# Autodesk Inventor assembly: Driveopen2
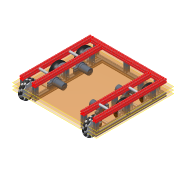
[picture p0: Inventor's stored thumbnail of the model, 180x180]
Saved by Autodesk Inventor 2013 (Build 170138000, 138)
## iProperties
Created: 2013-09-22
Part Number: Driveopen2
Document SubType Name: Assembly
Designer: Family Room
Mass: 858.54 g
Surface Area: 8628.43 cm^2
Volume: 788.69 cm^3
Density: 1.08856 g/cm^3
Author: Family Room
## Documents named in this file (14)
- H:\Driveopen2.iam
- H:\Frame Layer open.iam
- H:\Verticle support.ipt
- C:\Users\Family Room\Documents\Inventor\Content Center Files\R2011\en-US\ANSI B18.3(13)\ANSI B18.3 - 1_4-28 UNF - 1(22).ipt
- H:\axel support.ipt
- H:\Tetrix Wheel 4 in omni.ipt
- H:\Tetrix wheel 4 in.ipt
- H:\pvc holder.ipt
- C:\Users\rihoobler\Documents\Inventor\tetrix_739091_2012.ipt
- U:\Imported Components\tetrix_739088_2012\tetrix_739088_2012.ipt
- U:\Imported Components\tetrix_739165_2012\tetrix_739165_2012.ipt
- U:\Imported Components\tetrix_739172_2012\tetrix_739172_2012.iam
- H:\Motor Mount.ipt
- H:\Motor.iam
## Components (81 placed, 13 different names)
1. Frame Layer open:1 [sub-assembly] — Mate:3, Flush:5, Mate:4, Flush:6, Flush:9, Mate:6, Flush:11, Insert:4, Insert:5, Insert:6, Mate:12, Flush:12, Flush:13, Mate:13, Flush:14, Flush:15, Mate:14, Flush:16, Flush:17, Mate:15, Angle:1, Flush:18, Mate:17, Angle:2, Mate:18, Mate:19, Flush:19, Mate:20, Flush:21, Mate:21, Flush:23, Flush:24, Mate:22, Flush:25, Mate:23, Flush:27, Mate:24, Flush:29, Mate:25, Flush:31, Mate:32, Mate:35, Mate:37, Mate:38, Flush:44, Mate:72, Flush:50, Mate:74, Flush:51, Mate:76, Flush:52, Flush:53, Mate:77, Flush:60
2. Frame Layer open:2 [sub-assembly] — Flush:9, Flush:10, Insert:1, Insert:2, Insert:3, Mate:33, Mate:34, Mate:36, Mate:39
3. Verticle support:3 — Mate:4, Flush:6, Flush:10, Mate:7, Mate:10
4. Verticle support:4 — Mate:3, Flush:5, Mate:11
5. Verticle support:5 — Mate:6, Flush:11, Mate:7
6. Spline Socket Head Cap Screw - Inch 1/4-28 UNF - 1:1 — Insert:1
7. Spline Socket Head Cap Screw - Inch 1/4-28 UNF - 1:2 — Insert:2
8. Spline Socket Head Cap Screw - Inch 1/4-28 UNF - 1:3 — Insert:3
9. Spline Socket Head Cap Screw - Inch 1/4-28 UNF - 1:4 — Insert:4, Mate:10
10. Spline Socket Head Cap Screw - Inch 1/4-28 UNF - 1:5 — Insert:5
11. Spline Socket Head Cap Screw - Inch 1/4-28 UNF - 1:6 — Insert:6, Mate:11
12. axel support:1 — Mate:14, Flush:16, Flush:17, Mate:27, Insert:7
13. axel support:2 — Mate:25, Flush:31, Flush:32, Mate:31, Mate:48, Flush:43
14. axel support:3 — Mate:21, Flush:23, Flush:24, Mate:46, Mate:49, Flush:41
15. axel support:4 — Mate:12, Flush:12, Flush:13, Mate:16, Mate:26, Insert:10
16. axel support:5 — Mate:13, Flush:14, Flush:15, Insert:11, Flush:40
17. axel support:6 — Mate:15, Angle:1, Flush:18, Mate:16, Flush:20, Flush:26, Mate:28, Insert:14, Mate:73
18. axel support:7 — Mate:17, Angle:2, Mate:18, Flush:22, Flush:28, Mate:29, Insert:15, Mate:75
19. axel support:8 — Mate:19, Flush:19, Flush:20, Insert:12
20. axel support:9 — Mate:20, Flush:21, Flush:22, Insert:13
21. axel support:10 — Mate:24, Flush:29, Flush:30, Mate:30, Mate:47, Flush:42
22. axel support:11 — Mate:22, Flush:25, Flush:26, Flush:30, Insert:8
23. axel support:12 — Mate:23, Flush:27, Flush:28, Flush:32, Insert:9
24. Tetrix Wheel 4 in omni:1 — Mate:26, Mate:40, Mate:42, Mate:43, Flush:36, Insert:19
25. Tetrix Wheel 4 in omni:2 — Mate:27, Mate:41, Mate:44, Mate:45, Insert:24
26. Tetrix wheel 4 in:1 — Mate:31, Flush:34, Insert:26
27. Tetrix wheel 4 in:2 — Mate:30, Flush:34, Flush:35, Insert:25
28. Tetrix wheel 4 in:3 — Mate:28, Flush:36, Flush:37, Insert:21
29. Tetrix wheel 4 in:4 — Mate:29, Flush:37, Insert:22
30. pvc holder:1 — Mate:36
31. pvc holder:2 — Mate:39
32. pvc holder:3 — Mate:38
33. pvc holder:4 — Mate:37
34. pvc holder:5 — Mate:33
35. pvc holder:6 — Mate:32
36. pvc holder:7 — Mate:34
37. pvc holder:8 — Mate:35
38. Tetrix Wheel 4 in omni:3 — Mate:40, Mate:42, Mate:43, Insert:20
39. Tetrix Wheel 4 in omni:4 — Mate:41, Mate:44, Mate:45, Flush:35, Insert:27
40. tetrix_739091_2012:1 — Insert:10, Mate:50
41. tetrix_739091_2012:2 — Insert:11, Mate:61
42. tetrix_739091_2012:3 — Insert:12
43. tetrix_739091_2012:4 — Insert:14, Mate:51
44. tetrix_739091_2012:5 — Insert:15, Mate:52
45. tetrix_739091_2012:6 — Insert:13
46. tetrix_739091_2012:7 — Insert:7
47. tetrix_739091_2012:8 — Mate:46, Flush:38, Mate:49, Mate:53
48. tetrix_739091_2012:9 — Insert:8
49. tetrix_739091_2012:10 — Mate:47, Flush:38, Flush:39, Mate:54
50. tetrix_739091_2012:11 — Insert:9
51. tetrix_739091_2012:12 — Mate:48, Flush:39, Mate:55, Mate:67
52. tetrix_739088_2012:1 — Mate:50, Flush:40
53. tetrix_739088_2012:2 — Mate:51, Flush:44, Flush:45, Mate:60
54. tetrix_739088_2012:3 — Mate:52, Flush:45, Mate:65
55. tetrix_739088_2012:4 — Mate:53, Flush:41
56. tetrix_739088_2012:5 — Mate:54, Flush:42, Mate:68, Mate:69
57. tetrix_739088_2012:6 — Mate:55, Flush:43, Mate:71
58. tetrix_739165_2012:1 — Insert:19, Flush:46
59. tetrix_739165_2012:2 — Mate:63, Mate:64, Mate:66, Flush:47
60. tetrix_739165_2012:3 — Mate:60, Flush:46, Mate:63, Mate:64, Insert:23
61. tetrix_739165_2012:4 — Mate:68, Flush:48, Insert:28
62. tetrix_739165_2012:5 — Insert:27, Flush:48
63. tetrix_739165_2012:6 — Mate:65, Flush:47
64. tetrix_739172_2012:1 [sub-assembly] — Insert:20, Mate:61
65. tetrix_739172_2012:2 [sub-assembly] — Insert:21
66. tetrix_739172_2012:3 [sub-assembly] — Insert:22
67. tetrix_739172_2012:4 [sub-assembly] — Insert:23, Mate:66
68. tetrix_739172_2012:5 [sub-assembly] — Insert:26, Mate:67
69. tetrix_739172_2012:6 [sub-assembly] — Insert:25
70. tetrix_739172_2012:7 [sub-assembly] — Insert:24
71. tetrix_739172_2012:8 [sub-assembly] — Insert:28, Mate:70
72. tetrix_739165_2012:7 — Mate:71, Flush:49
73. tetrix_739165_2012:8 — Mate:69, Mate:70, Flush:49
74. Motor Mount:1 — Mate:72, Flush:50, Mate:73, Flush:55, Mate:78, Flush:57
75. Motor Mount:2 — Mate:74, Flush:51, Mate:75, Flush:54, Mate:79, Flush:56
76. Motor Mount:3 — Mate:76, Flush:52, Flush:55, Mate:80, Flush:58
77. Motor Mount:4 — Flush:53, Mate:77, Flush:54, Mate:81, Flush:59
78. Motor:1 [sub-assembly] — Mate:78, Flush:57
79. Motor:2 [sub-assembly] — Mate:79, Flush:56
80. Motor:3 [sub-assembly] — Mate:80, Flush:58
81. Motor:4 [sub-assembly] — Mate:81, Flush:59
## Relationships (153: Mate 71, Flush 55, Insert 25, Angle 2)
- Mate:3: Frame Layer open:1 ↔ Verticle support:4
- Flush:5: Frame Layer open:1 ↔ Verticle support:4
- Mate:4: Frame Layer open:1 ↔ Verticle support:3
- Flush:6: Frame Layer open:1 ↔ Verticle support:3
- Flush:9: Frame Layer open:1 ↔ Frame Layer open:2
- Flush:10: Frame Layer open:2 ↔ Verticle support:3
- Mate:6: Frame Layer open:1 ↔ Verticle support:5
- Flush:11: Frame Layer open:1 ↔ Verticle support:5
- Mate:7 (156.8526 mm): Verticle support:3 ↔ Verticle support:5
- Insert:1: Frame Layer open:2 ↔ Spline Socket Head Cap Screw - Inch 1/4-28 UNF - 1:1
- Insert:2: Frame Layer open:2 ↔ Spline Socket Head Cap Screw - Inch 1/4-28 UNF - 1:2
- Insert:3: Frame Layer open:2 ↔ Spline Socket Head Cap Screw - Inch 1/4-28 UNF - 1:3
- Insert:4: Frame Layer open:1 ↔ Spline Socket Head Cap Screw - Inch 1/4-28 UNF - 1:4
- Insert:5: Frame Layer open:1 ↔ Spline Socket Head Cap Screw - Inch 1/4-28 UNF - 1:5
- Insert:6: Frame Layer open:1 ↔ Spline Socket Head Cap Screw - Inch 1/4-28 UNF - 1:6
- Mate:10: Verticle support:3 ↔ Spline Socket Head Cap Screw - Inch 1/4-28 UNF - 1:4
- Mate:11: Verticle support:4 ↔ Spline Socket Head Cap Screw - Inch 1/4-28 UNF - 1:6
- Mate:12: Frame Layer open:1 ↔ axel support:4
- Flush:12: Frame Layer open:1 ↔ axel support:4
- Flush:13: Frame Layer open:1 ↔ axel support:4
- Mate:13: Frame Layer open:1 ↔ axel support:5
- Flush:14: Frame Layer open:1 ↔ axel support:5
- Flush:15: Frame Layer open:1 ↔ axel support:5
- Mate:14: Frame Layer open:1 ↔ axel support:1
- Flush:16: Frame Layer open:1 ↔ axel support:1
- Flush:17: Frame Layer open:1 ↔ axel support:1
- Mate:15: Frame Layer open:1 ↔ axel support:6
- Angle:1 (0 deg): Frame Layer open:1 ↔ axel support:6
- Flush:18: Frame Layer open:1 ↔ axel support:6
- Mate:16 (158.75 mm): axel support:4 ↔ axel support:6
- Mate:17: Frame Layer open:1 ↔ axel support:7
- Angle:2 (0 deg): Frame Layer open:1 ↔ axel support:7
- Mate:18: Frame Layer open:1 ↔ axel support:7
- Mate:19: Frame Layer open:1 ↔ axel support:8
- Flush:19: Frame Layer open:1 ↔ axel support:8
- Flush:20: axel support:6 ↔ axel support:8
- Mate:20: Frame Layer open:1 ↔ axel support:9
- Flush:21: Frame Layer open:1 ↔ axel support:9
- Flush:22: axel support:7 ↔ axel support:9
- Mate:21: Frame Layer open:1 ↔ axel support:3
- Flush:23: Frame Layer open:1 ↔ axel support:3
- Flush:24: Frame Layer open:1 ↔ axel support:3
- Mate:22: Frame Layer open:1 ↔ axel support:11
- Flush:25: Frame Layer open:1 ↔ axel support:11
- Flush:26: axel support:6 ↔ axel support:11
- Mate:23: Frame Layer open:1 ↔ axel support:12
- Flush:27: Frame Layer open:1 ↔ axel support:12
- Flush:28: axel support:7 ↔ axel support:12
- Mate:24: Frame Layer open:1 ↔ axel support:10
- Flush:29: Frame Layer open:1 ↔ axel support:10
- Flush:30: axel support:10 ↔ axel support:11
- Mate:25: Frame Layer open:1 ↔ axel support:2
- Flush:31: Frame Layer open:1 ↔ axel support:2
- Flush:32: axel support:2 ↔ axel support:12
- Mate:26: axel support:4 ↔ Tetrix Wheel 4 in omni:1
- Mate:27: axel support:1 ↔ Tetrix Wheel 4 in omni:2
- Mate:28: axel support:6 ↔ Tetrix wheel 4 in:3
- Mate:29: axel support:7 ↔ Tetrix wheel 4 in:4
- Mate:30: axel support:10 ↔ Tetrix wheel 4 in:2
- Mate:31: axel support:2 ↔ Tetrix wheel 4 in:1
- Mate:32: Frame Layer open:1 ↔ pvc holder:6
- Mate:33: Frame Layer open:2 ↔ pvc holder:5
- Mate:34: Frame Layer open:2 ↔ pvc holder:7
- Mate:35: Frame Layer open:1 ↔ pvc holder:8
- Mate:36: Frame Layer open:2 ↔ pvc holder:1
- Mate:37: Frame Layer open:1 ↔ pvc holder:4
- Mate:38: Frame Layer open:1 ↔ pvc holder:3
- Mate:39: Frame Layer open:2 ↔ pvc holder:2
- Mate:40: Tetrix Wheel 4 in omni:1 ↔ Tetrix Wheel 4 in omni:3
- Mate:41: Tetrix Wheel 4 in omni:2 ↔ Tetrix Wheel 4 in omni:4
- Mate:42: Tetrix Wheel 4 in omni:1 ↔ Tetrix Wheel 4 in omni:3
- Mate:43: Tetrix Wheel 4 in omni:1 ↔ Tetrix Wheel 4 in omni:3
- Mate:44: Tetrix Wheel 4 in omni:2 ↔ Tetrix Wheel 4 in omni:4
- Mate:45: Tetrix Wheel 4 in omni:2 ↔ Tetrix Wheel 4 in omni:4
- Flush:34: Tetrix wheel 4 in:1 ↔ Tetrix wheel 4 in:2
- Flush:35: Tetrix wheel 4 in:2 ↔ Tetrix Wheel 4 in omni:4
- Flush:36: Tetrix Wheel 4 in omni:1 ↔ Tetrix wheel 4 in:3
- Flush:37: Tetrix wheel 4 in:3 ↔ Tetrix wheel 4 in:4
- Mate:46: axel support:3 ↔ tetrix_739091_2012:8
- Mate:47: axel support:10 ↔ tetrix_739091_2012:10
- Flush:38: tetrix_739091_2012:8 ↔ tetrix_739091_2012:10
- Mate:48: axel support:2 ↔ tetrix_739091_2012:12
- Flush:39: tetrix_739091_2012:10 ↔ tetrix_739091_2012:12
- Mate:49: axel support:3 ↔ tetrix_739091_2012:8
- Insert:7: axel support:1 ↔ tetrix_739091_2012:7
- Insert:8: axel support:11 ↔ tetrix_739091_2012:9
- Insert:9: axel support:12 ↔ tetrix_739091_2012:11
- Insert:10: axel support:4 ↔ tetrix_739091_2012:1
- Insert:11: axel support:5 ↔ tetrix_739091_2012:2
- Insert:12: axel support:8 ↔ tetrix_739091_2012:3
- Insert:13: axel support:9 ↔ tetrix_739091_2012:6
- Insert:14: axel support:6 ↔ tetrix_739091_2012:4
- Insert:15: axel support:7 ↔ tetrix_739091_2012:5
- Mate:50: tetrix_739091_2012:1 ↔ tetrix_739088_2012:1
- Flush:40: axel support:5 ↔ tetrix_739088_2012:1
- Mate:51: tetrix_739091_2012:4 ↔ tetrix_739088_2012:2
- Mate:52: tetrix_739091_2012:5 ↔ tetrix_739088_2012:3
- Mate:53: tetrix_739091_2012:8 ↔ tetrix_739088_2012:4
- Mate:54: tetrix_739091_2012:10 ↔ tetrix_739088_2012:5
- Mate:55: tetrix_739091_2012:12 ↔ tetrix_739088_2012:6
- Flush:41: axel support:3 ↔ tetrix_739088_2012:4
- Flush:42: axel support:10 ↔ tetrix_739088_2012:5
- Flush:43: axel support:2 ↔ tetrix_739088_2012:6
- Flush:44: Frame Layer open:1 ↔ tetrix_739088_2012:2
- Flush:45: tetrix_739088_2012:2 ↔ tetrix_739088_2012:3
- Insert:19: Tetrix Wheel 4 in omni:1 ↔ tetrix_739165_2012:1
- Mate:60: tetrix_739088_2012:2 ↔ tetrix_739165_2012:3
- Flush:46: tetrix_739165_2012:1 ↔ tetrix_739165_2012:3
- Insert:20: Tetrix Wheel 4 in omni:3 ↔ tetrix_739172_2012:1
- Mate:61: tetrix_739091_2012:2 ↔ tetrix_739172_2012:1
- Insert:21: Tetrix wheel 4 in:3 ↔ tetrix_739172_2012:2
- Insert:22: Tetrix wheel 4 in:4 ↔ tetrix_739172_2012:3
- Mate:63: tetrix_739165_2012:2 ↔ tetrix_739165_2012:3
- Mate:64: tetrix_739165_2012:2 ↔ tetrix_739165_2012:3
- Mate:65: tetrix_739088_2012:3 ↔ tetrix_739165_2012:6
- Insert:23: tetrix_739165_2012:3 ↔ tetrix_739172_2012:4
- Mate:66: tetrix_739165_2012:2 ↔ tetrix_739172_2012:4
- Flush:47: tetrix_739165_2012:2 ↔ tetrix_739165_2012:6
- Insert:24: Tetrix Wheel 4 in omni:2 ↔ tetrix_739172_2012:7
- Insert:25: Tetrix wheel 4 in:2 ↔ tetrix_739172_2012:6
- Insert:26: Tetrix wheel 4 in:1 ↔ tetrix_739172_2012:5
- Mate:67: tetrix_739091_2012:12 ↔ tetrix_739172_2012:5
- Insert:27: Tetrix Wheel 4 in omni:4 ↔ tetrix_739165_2012:5
- Mate:68: tetrix_739088_2012:5 ↔ tetrix_739165_2012:4
- Flush:48: tetrix_739165_2012:4 ↔ tetrix_739165_2012:5
- Insert:28: tetrix_739165_2012:4 ↔ tetrix_739172_2012:8
- Mate:69: tetrix_739088_2012:5 ↔ tetrix_739165_2012:8
- Mate:70: tetrix_739172_2012:8 ↔ tetrix_739165_2012:8
- Mate:71: tetrix_739088_2012:6 ↔ tetrix_739165_2012:7
- Flush:49: tetrix_739165_2012:7 ↔ tetrix_739165_2012:8
- Mate:72: Frame Layer open:1 ↔ Motor Mount:1
- Flush:50: Frame Layer open:1 ↔ Motor Mount:1
- Mate:73 (25.4 mm): axel support:6 ↔ Motor Mount:1
- Mate:74: Frame Layer open:1 ↔ Motor Mount:2
- Flush:51: Frame Layer open:1 ↔ Motor Mount:2
- Mate:75 (25.4 mm): axel support:7 ↔ Motor Mount:2
- Mate:76: Frame Layer open:1 ↔ Motor Mount:3
- Flush:52: Frame Layer open:1 ↔ Motor Mount:3
- Flush:53: Frame Layer open:1 ↔ Motor Mount:4
- Mate:77: Frame Layer open:1 ↔ Motor Mount:4
- Flush:54: Motor Mount:2 ↔ Motor Mount:4
- Flush:55: Motor Mount:1 ↔ Motor Mount:3
- Mate:78: Motor Mount:1 ↔ Motor:1
- Mate:79: Motor Mount:2 ↔ Motor:2
- Mate:80: Motor Mount:3 ↔ Motor:3
- Mate:81: Motor Mount:4 ↔ Motor:4
- Flush:56: Motor Mount:2 ↔ Motor:2
- Flush:57: Motor Mount:1 ↔ Motor:1
- Flush:58: Motor Mount:3 ↔ Motor:3
- Flush:59: Motor Mount:4 ↔ Motor:4
- Flush:60 (12.7 mm): Frame Layer open:1
- Flush:61 (17.907 mm)
- Flush:62 (-17.907 mm)
